# Autodesk Inventor assembly: Leg_Right
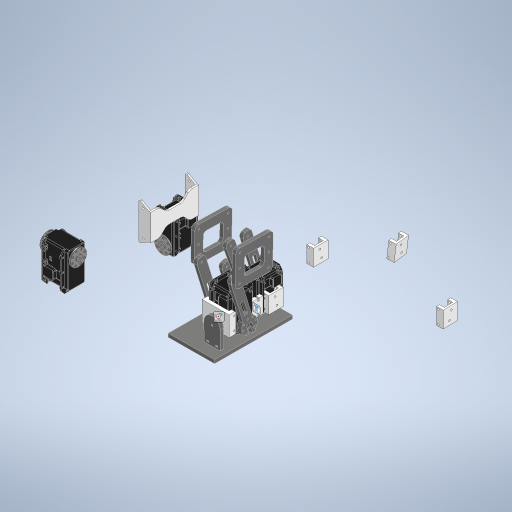
[picture p0: Inventor's stored thumbnail of the model, 512x512]
Saved by Autodesk Inventor 2024.3 (Build 283343000, 343)
## iProperties
Created: 2024-09-18
Part Number: Leg_Right
Document SubType Name: Assembly
Designer: 구지현
Author: 구지현
## Documents named in this file (20)
- C:\Users\구지현\Desktop\19th_intern_kdy_robot\부품\Lower_Body\Leg\Leg_Right.iam
- C:\Users\구지현\Documents\카카오톡 받은 파일\Hardware\ROBOTIS(Inventor 2024 ver.)\다이나믹셀\MX-64T+idle.ipt.iam
- C:\Users\구지현\Documents\카카오톡 받은 파일\Hardware\ROBOTIS(Inventor 2024 ver.)\다이나믹셀\MX-106T+idle.ipt.iam
- C:\Users\구지현\Documents\카카오톡 받은 파일\Hardware\ROBOTIS(Inventor 2024 ver.)\혼\64-106Horn.ipt
- C:\Users\구지현\Desktop\19th_intern_kdy_robot\부품\Lower_Body\Leg\Back_Ankle.ipt
- C:\Users\구지현\Desktop\19th_intern_kdy_robot\부품\Lower_Body\Leg\Foot_MIR.ipt
- C:\Users\구지현\Desktop\19th_intern_kdy_robot\부품\Lower_Body\Leg\Front_Ankle.ipt
- C:\Users\구지현\Desktop\19th_intern_kdy_robot\부품\Lower_Body\Leg\Knee.ipt
- C:\Users\구지현\Desktop\19th_intern_kdy_robot\부품\Lower_Body\Leg\Knee_Covers.ipt
- C:\Users\구지현\Desktop\19th_intern_kdy_robot\부품\Lower_Body\Leg\Leg_Connection_Parts_Back.ipt
- C:\Users\구지현\Desktop\19th_intern_kdy_robot\부품\Lower_Body\Leg\Leg_Connection_Parts_Front.ipt
- C:\Users\구지현\Desktop\19th_intern_kdy_robot\부품\Lower_Body\Leg\Leg_Foot_Connection_Parts.ipt
- C:\Users\구지현\Desktop\19th_intern_kdy_robot\부품\Lower_Body\Leg\Link_Fixation_Connector.ipt
- C:\Users\구지현\Desktop\19th_intern_kdy_robot\부품\Lower_Body\Leg\Link_Fixation_Connector_MIR.ipt
- Link_Fixation_Connector_left_left.ipt
- C:\Users\구지현\Desktop\19th_intern_kdy_robot\부품\Lower_Body\Leg\Link_Fixation_Connector_MIR_MIR.ipt
- C:\Users\구지현\Desktop\19th_intern_kdy_robot\부품\Lower_Body\Leg\Link_Fixation_Connector_MIR1.ipt
- C:\Users\구지현\Desktop\19th_intern_kdy_robot\부품\Lower_Body\Leg\Vertical_Fixation_Set.iam
- MX-106T+idle.ipt
- MX-64T+idle.ipt
## Components (27 placed, 16 different names)
1. MX-106T+idle.ipt:3 [sub-assembly]
2. 64-106Horn:5
3. MX-106T+idle.ipt:4 [sub-assembly] — 메이트:1, 메이트:2, 메이트:3, 메이트:6, 메이트:7, 메이트:8, 메이트:10, 메이트:11
4. 64-106Horn:6 — 메이트:12, 메이트:13
5. MX-64T+idle.ipt:3 [sub-assembly]
6. 64-106Horn:7
7. MX-64T+idle.ipt:4 [sub-assembly] — 삽입:12, 메이트:9, 메이트:14, 메이트:15, 메이트:16, 메이트:18, 메이트:19, 메이트:20
8. 64-106Horn:8 — 삽입:10
9. Back_Ankle:1 — 삽입:10, 플러쉬:1, 각도:1, 삽입:14
10. Foot_MIR:1 — 삽입:13, 삽입:14
11. Front_Ankle:1 — 삽입:11, 플러쉬:1, 각도:1, 삽입:13
12. Knee:1 — 삽입:15, 삽입:16
13. Knee_Covers:1
14. Leg_Connection_Parts_Front:1 — 메이트:12, 메이트:13, 플러쉬:2, 플러쉬:3, 플러쉬:5, 삽입:15
15. Leg_Foot_Connection_Parts:1 — 메이트:6, 메이트:7, 메이트:8, 삽입:11
16. Link_Fixation_Connector:1 — 메이트:14, 메이트:15, 메이트:16
17. Link_Fixation_Connector_left_left:1
18. Link_Fixation_Connector_MIR_MIR:1
19. Vertical_Fixation_Set:1 [sub-assembly] — 메이트:1, 메이트:2, 메이트:3, 삽입:12, 메이트:9
20. Leg_Connection_Parts_Front:2 — 메이트:10, 메이트:11, 플러쉬:2, 플러쉬:3, 삽입:17
21. Leg_Connection_Parts_Back:3 — 메이트:21, 플러쉬:5, 삽입:16
22. Link_Fixation_Connector_MIR1:2
23. Link_Fixation_Connector_MIR1:3 — 메이트:18, 메이트:19, 메이트:20, 메이트:21
24. Leg_Connection_Parts_Back:4
25. Leg_Connection_Parts_Back:5
26. Knee:2 — 삽입:17
27. Link_Fixation_Connector:2
## Relationships (35: Mate 18, Insert 12, Flush 4, Angle 1)
- [Insert]: MX-106T+idle.ipt:3 ↔ 64-106Horn:5
- [Insert]: MX-106T+idle.ipt:4 ↔ 64-106Horn:6
- [Insert]: MX-64T+idle.ipt:3 ↔ 64-106Horn:7
- [Insert]: MX-64T+idle.ipt:4 ↔ 64-106Horn:8
- 메이트:1 [Mate] (0.1 mm): MX-106T+idle.ipt:4 ↔ Vertical_Fixation_Set:1
- 메이트:2 [Mate]: MX-106T+idle.ipt:4 ↔ Vertical_Fixation_Set:1
- 메이트:3 [Mate]: MX-106T+idle.ipt:4 ↔ Vertical_Fixation_Set:1
- 삽입:10 [Insert]: 64-106Horn:8 ↔ Back_Ankle:1
- 메이트:6 [Mate]: MX-106T+idle.ipt:4 ↔ Leg_Foot_Connection_Parts:1
- 메이트:7 [Mate] (0.1 mm): MX-106T+idle.ipt:4 ↔ Leg_Foot_Connection_Parts:1
- 메이트:8 [Mate]: MX-106T+idle.ipt:4 ↔ Leg_Foot_Connection_Parts:1
- 삽입:11 [Insert]: Front_Ankle:1 ↔ Leg_Foot_Connection_Parts:1
- 삽입:12 [Insert]: MX-64T+idle.ipt:4 ↔ Vertical_Fixation_Set:1
- 메이트:9 [Mate]: MX-64T+idle.ipt:4 ↔ Vertical_Fixation_Set:1
- 플러쉬:1 [Flush]: Back_Ankle:1 ↔ Front_Ankle:1
- 각도:1 [Angle] (0 deg): Back_Ankle:1 ↔ Front_Ankle:1
- 삽입:13 [Insert]: Foot_MIR:1 ↔ Front_Ankle:1
- 삽입:14 [Insert]: Back_Ankle:1 ↔ Foot_MIR:1
- 메이트:10 [Mate]: MX-106T+idle.ipt:4 ↔ Leg_Connection_Parts_Front:2
- 메이트:11 [Mate]: MX-106T+idle.ipt:4 ↔ Leg_Connection_Parts_Front:2
- 메이트:12 [Mate]: 64-106Horn:6 ↔ Leg_Connection_Parts_Front:1
- 메이트:13 [Mate]: 64-106Horn:6 ↔ Leg_Connection_Parts_Front:1
- 플러쉬:2 [Flush]: Leg_Connection_Parts_Front:1 ↔ Leg_Connection_Parts_Front:2
- 플러쉬:3 [Flush]: Leg_Connection_Parts_Front:1 ↔ Leg_Connection_Parts_Front:2
- 메이트:14 [Mate] (0.1 mm): MX-64T+idle.ipt:4 ↔ Link_Fixation_Connector:1
- 메이트:15 [Mate]: MX-64T+idle.ipt:4 ↔ Link_Fixation_Connector:1
- 메이트:16 [Mate]: MX-64T+idle.ipt:4 ↔ Link_Fixation_Connector:1
- 메이트:18 [Mate]: MX-64T+idle.ipt:4 ↔ Link_Fixation_Connector_MIR1:3
- 메이트:19 [Mate]: MX-64T+idle.ipt:4 ↔ Link_Fixation_Connector_MIR1:3
- 메이트:20 [Mate]: MX-64T+idle.ipt:4 ↔ Link_Fixation_Connector_MIR1:3
- 메이트:21 [Mate]: Leg_Connection_Parts_Back:3 ↔ Link_Fixation_Connector_MIR1:3
- 플러쉬:5 [Flush]: Leg_Connection_Parts_Front:1 ↔ Leg_Connection_Parts_Back:3
- 삽입:15 [Insert]: Knee:1 ↔ Leg_Connection_Parts_Front:1
- 삽입:16 [Insert]: Knee:1 ↔ Leg_Connection_Parts_Back:3
- 삽입:17 [Insert]: Leg_Connection_Parts_Front:2 ↔ Knee:2
## Named parameters: d7_d130 = 0 mm, d8_d0_d1 = 0 mm, d9_d118 = 0 mm, d10_d140 = 0 mm
